# Autodesk Inventor assembly: konsol
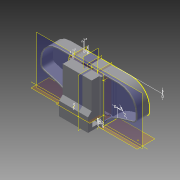
[picture p0: Inventor's stored thumbnail of the model, 180x180]
Saved by Autodesk Inventor 2015 (Build 190159000, 159)
## iProperties
Created: 2015-12-13
Part Number: konsol
Document SubType Name: Assembly
Designer: abberik
Mass: 114.13 g
Surface Area: 1187.84 cm^2
Volume: 114.13 cm^3
Density: 1 g/cm^3
Author: abberik
## Documents named in this file (5)
- E:\bibliotek\dokument\Raspberry Pi gaming konsol\konsol.iam
- E:\bibliotek\dokument\Raspberry Pi gaming konsol\kontroller3.ipt
- E:\bibliotek\dokument\Raspberry Pi gaming konsol\PI_Skal_med_rals.ipt
- E:\bibliotek\dokument\Raspberry Pi gaming konsol\batteri.ipt
- E:\bibliotek\dokument\Raspberry Pi gaming konsol\batterilock.ipt
## Components (4 placed, 4 different names)
1. kontroller3:1 — Mate:1, Mate:2, Flush:1, Mate:4, Mate:5
2. PI_Skal_med_rals:1 — Mate:1, Mate:2, Flush:1, Mate:3
3. batteri:1 — Mate:3, Mate:4, Mate:5, Mate:6, Mate:7, Mate:8
4. batterilock:1 — Mate:6, Mate:7, Mate:8
## Relationships (9: Mate 8, Flush 1)
- Mate:1: kontroller3:1 ↔ PI_Skal_med_rals:1
- Mate:2: kontroller3:1 ↔ PI_Skal_med_rals:1
- Flush:1: kontroller3:1 ↔ PI_Skal_med_rals:1
- Mate:3: PI_Skal_med_rals:1 ↔ batteri:1
- Mate:4: kontroller3:1 ↔ batteri:1
- Mate:5: kontroller3:1 ↔ batteri:1
- Mate:6: batteri:1 ↔ batterilock:1
- Mate:7: batteri:1 ↔ batterilock:1
- Mate:8: batteri:1 ↔ batterilock:1
